# Autodesk Inventor assembly: 4Wire-FDM-Pivot
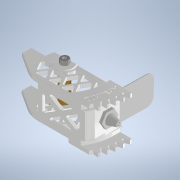
[picture p0: Inventor's stored thumbnail of the model, 180x180]
Saved by Autodesk Inventor 2021 (Build 250183000, 183)
## iProperties
Created: 2020-08-18
Part Number: 4Wire-FDM-Pivot
Document SubType Name: Assembly
Designer: lucas
Author: lucas
## Documents named in this file (9)
- C:\Users\lucas\Nextcloud\HackerSpace\HV Home Battery Storage Project\Concepts & Storyboards\18650 4wire Holder\4Wire-FDM-Slot\4Wire-FDM-Pivot.iam
- C:\Users\lucas\Nextcloud\HackerSpace\HV Home Battery Storage Project\Concepts & Storyboards\18650 4wire Holder\4Wire-FDM-Slot\FDM-Pivot.ipt
- C:\Users\lucas\Nextcloud\HackerSpace\HV Home Battery Storage Project\Concepts & Storyboards\18650 4wire Holder\4Wire-FDM-Slot\Standoff-M3x20mm.ipt
- C:\Users\lucas\Documents\Inventor\Content Center Files\R2021\en-US\ISO 4762(2)\ISO 4762 - M3 x 6ISO.ipt
- C:\Users\lucas\Nextcloud\HackerSpace\HV Home Battery Storage Project\Concepts & Storyboards\18650 4wire Holder\ZKE\ZKE-Term-Solid.ipt
- C:\Users\lucas\Nextcloud\HackerSpace\HV Home Battery Storage Project\Concepts & Storyboards\18650 4wire Holder\4Wire-FDM-Slot\FDM-Pivot-Ringpull.ipt
- C:\Users\lucas\Nextcloud\HackerSpace\HV Home Battery Storage Project\Concepts & Storyboards\18650 4wire Holder\ZKE\ZKE-Term-Solid-Shim.ipt
- C:\Users\lucas\Nextcloud\HackerSpace\HV Home Battery Storage Project\Concepts & Storyboards\18650 4wire Holder\Shared Parts\Pogo_pin_P75-E2.ipt
- C:\Users\lucas\Documents\Inventor\Content Center Files\R2021\en-US\ISO 4035(2)\ISO 4035 - M8 - ISO.ipt
## Components (9 placed, 8 different names)
1. FDM-Pivot:1 — Rotational:1, Insert:1, Insert:2, Rotational:5, Rotational:6, Rotational:7
2. Shaft:1 — Rotational:1
3. ISO 4762 M3 x 6:1 — Insert:1
4. ISO 4762 M3 x 6:2 — Insert:2
5. ZKE-Term-Solid:1 — Rigid:1, Rotational:5
6. FDM-Pivot-Ringpull:1 — Rotational:6
7. ZKE-Term-Solid-Shim:1 — Rotational:7
8. Pogo_pin_P75-E2:1 — Rigid:1
9. ISO 4035 M8:1
## Relationships (8: RevoluteJoint 4, Insert 3, WeldJoint 1)
- Rotational:1 [RevoluteJoint]: FDM-Pivot:1 ↔ Shaft:1
- Insert:1: FDM-Pivot:1 ↔ ISO 4762 M3 x 6:1
- Insert:2: FDM-Pivot:1 ↔ ISO 4762 M3 x 6:2
- Rigid:1 [WeldJoint]: ZKE-Term-Solid:1 ↔ Pogo_pin_P75-E2:1
- Rotational:5 [RevoluteJoint]: FDM-Pivot:1 ↔ ZKE-Term-Solid:1
- Rotational:6 [RevoluteJoint]: FDM-Pivot:1 ↔ FDM-Pivot-Ringpull:1
- Rotational:7 [RevoluteJoint]: FDM-Pivot:1 ↔ ZKE-Term-Solid-Shim:1
- [Insert]: ZKE-Term-Solid-Shim:1 ↔ ISO 4035 M8:1
